# Autodesk Inventor assembly: тело фулл
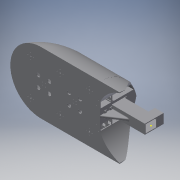
[picture p0: Inventor's stored thumbnail of the model, 180x180]
Saved by Autodesk Inventor 2019 (Build 230136000, 136)
## iProperties
Created: 2019-09-06
Part Number: тело фулл
Material: Типовые
Document SubType Name: Assembly
Designer: Iliga
Author: Iliga
## Documents named in this file (7)
- C:\Users\Iliga\Desktop\Robot\RobotFix1\робот\тело фулл.iam
- C:\Users\Iliga\Desktop\Robot\RobotFix1\робот\тело.ipt
- C:\Users\Iliga\Desktop\Robot\RobotFix1\робот\правое надкрылье.ipt
- C:\Users\Iliga\Desktop\Robot\RobotFix1\робот\полочка.ipt
- C:\Users\Iliga\Desktop\Robot\RobotFix1\робот\рога.ipt
- C:\Users\Iliga\Desktop\Robot\RobotFix1\робот\хребет2.ipt
- C:\Users\Iliga\Desktop\Robot\RobotFix1\робот\хребет.ipt
## Components (6 placed, 5 different names)
1. тело основа:1 — Заподлицо:3, Совмещение:2, Совмещение:3, Совмещение:4, Касательность:1, Заподлицо:4, Совмещение:6, Совмещение:7, Совмещение:8, Совмещение:10
2. правое надкрылье:1 — Заподлицо:3, Совмещение:2, Совмещение:3, Совмещение:5
3. полочка:2 — Совмещение:4, Касательность:1, Заподлицо:4
4. тело основа:3 — Совмещение:5, Совмещение:6, Совмещение:7
5. хребет2:4 — Совмещение:8, Заподлицо:5, Совмещение:9
6. хребет:1 — Совмещение:9, Совмещение:10, Совмещение:11
## Relationships (14: Mate 10, Flush 3, Tangent 1)
- Заподлицо:3 [Flush]: тело основа:1 ↔ правое надкрылье:1
- Совмещение:2 [Mate]: тело основа:1 ↔ правое надкрылье:1
- Совмещение:3 [Mate]: тело основа:1 ↔ правое надкрылье:1
- Совмещение:4 [Mate]: тело основа:1 ↔ полочка:2
- Касательность:1 [Tangent]: тело основа:1 ↔ полочка:2
- Заподлицо:4 [Flush]: тело основа:1 ↔ полочка:2
- Совмещение:5 [Mate]: правое надкрылье:1 ↔ тело основа:3
- Совмещение:6 [Mate]: тело основа:1 ↔ тело основа:3
- Совмещение:7 [Mate]: тело основа:1 ↔ тело основа:3
- Совмещение:8 [Mate]: тело основа:1 ↔ хребет2:4
- Заподлицо:5 [Flush]: хребет2:4
- Совмещение:9 [Mate]: хребет2:4 ↔ хребет:1
- Совмещение:10 [Mate]: тело основа:1 ↔ хребет:1
- Совмещение:11 [Mate]: хребет:1
